# Autodesk Inventor assembly: DayLightGlow_DisplayPanel_096
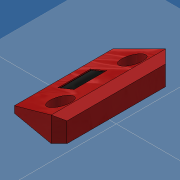
[picture p0: Inventor's stored thumbnail of the model, 180x180]
Saved by Autodesk Inventor 2019 (Build 230136000, 136)
## iProperties
Created: 2019-02-03
Part Number: DayLightGlow_DisplayPanel_096
Material: Generisch
Document SubType Name: Assembly
Designer: Stefan
Mass: 26.4034 g
Surface Area: 170.168 cm^2
Volume: 13.6862 cm^3
Density: 1.92919 g/cm^3
Author: Stefan
## Documents named in this file (3)
- C:\Users\User\Documents\Inventor\DayLightGlow\DayLightGlow_DisplayPanel_096.iam
- C:\Users\User\Documents\Inventor\DayLightGlow\DayLightGlow_DisplayPanel_096.ipt
- C:\Users\User\Documents\Inventor\DayLightGlow\LM096-128064 OLED DISPLAY .ipt
## Components (2 placed, 2 different names)
1. DayLightGlow_DisplayPanel_096:1 — Passend:1, Fluchtend:1
2. LM096-128064 OLED DISPLAY :1 — Passend:1, Fluchtend:1
## Relationships (2: Mate 1, Flush 1)
- Passend:1 [Mate]: DayLightGlow_DisplayPanel_096:1 ↔ LM096-128064 OLED DISPLAY :1
- Fluchtend:1 [Flush]: DayLightGlow_DisplayPanel_096:1 ↔ LM096-128064 OLED DISPLAY :1
